# Autodesk Inventor assembly: 전체 조립품
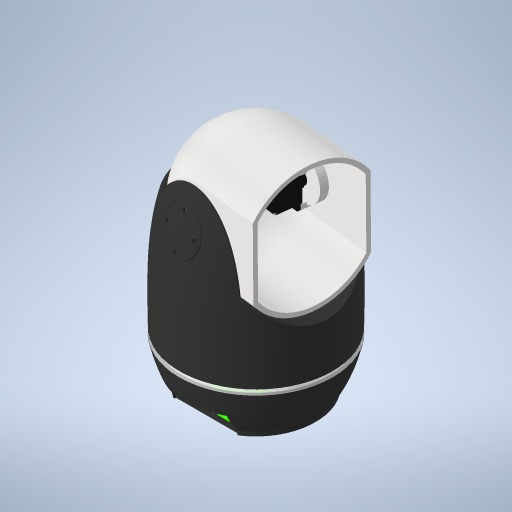
[picture p0: Inventor's stored thumbnail of the model, 512x512]
Saved by Autodesk Inventor 2023 (Build 270158000, 158)
## iProperties
Created: 2022-06-06
Part Number: 전체 조립품
Document SubType Name: Assembly
Designer: fly01
Author: fly01
## Documents named in this file (3)
- C:\Users\fly01\Desktop\2022카이스트 입학준비\스마트홈\제작부품'\전체 조립품.iam
- C:\Users\fly01\Desktop\2022카이스트 입학준비\스마트홈\제작부품'\상단부 조립품.iam
- C:\Users\fly01\Desktop\2022카이스트 입학준비\스마트홈\제작부품'\하단부 조립품.iam
## Components (2 placed, 2 different names)
1. 하단부 조립품:1 [sub-assembly] — 삽입:1
2. 상단부 조립품:2 [sub-assembly] — 삽입:1
## Relationships (1: Insert 1)
- 삽입:1 [Insert]: 하단부 조립품:1 ↔ 상단부 조립품:2
